# Autodesk Inventor assembly: FULL FINGE6
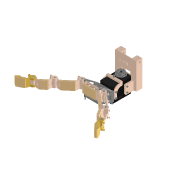
[picture p0: Inventor's stored thumbnail of the model, 180x180]
Saved by Autodesk Inventor 2021 (Build 250183000, 183)
## iProperties
Created: 2022-10-03
Part Number: FULL FINGE6
Document SubType Name: Assembly
Designer: ereg140
Author: ereg140
## Documents named in this file (21)
- \\files.auckland.ac.nz\myhome\Documents\GitHub\hand\FULL FINGE7.iam
- \\files.auckland.ac.nz\myhome\Documents\GitHub\hand\XM430 Motor\XM430-Working-Shaft.iam
- \\files.auckland.ac.nz\myhome\Documents\GitHub\hand\Dovetail\dovetail_female_Dyna_Mount.ipt
- \\files.auckland.ac.nz\myhome\Documents\GitHub\hand\Tendon_Center.ipt
- \\files.auckland.ac.nz\myhome\Documents\GitHub\hand\PLANGE7\Phalalnge7_HDM_45mm.ipt
- \\files.auckland.ac.nz\myhome\Documents\GitHub\hand\PLANGE7\Phalalnge7_HDM_35mm.ipt
- \\files.auckland.ac.nz\myhome\Documents\GitHub\hand\PLANGE7\Phalalnge7_35mm_TIP_hdm.ipt
- \\files.auckland.ac.nz\myhome\Documents\GitHub\hand\PLANGE7\FINGIE_7_palm_50mm.ipt
- \\files.auckland.ac.nz\myhome\Documents\GitHub\hand\Dynamixel_Palm_Bracket_3.ipt
- \\files.auckland.ac.nz\myhome\Documents\GitHub\hand\hardware\m2_18mm.ipt
- \\files.auckland.ac.nz\myhome\Documents\GitHub\hand\hardware\m2_40mm.ipt
- \\files.auckland.ac.nz\myhome\Documents\GitHub\hand\hardware\m2_nut.ipt
- \\files.auckland.ac.nz\myhome\Documents\GitHub\hand\hardware\M2_6mm.ipt
- \\files.auckland.ac.nz\myhome\Documents\GitHub\hand\hardware\M2_5_6mm.ipt
- \\files.auckland.ac.nz\myhome\Documents\GitHub\hand\Pully_smallest.ipt
- \\files.auckland.ac.nz\myhome\Documents\GitHub\hand\hardware\M2_3mm.ipt
- \\files.auckland.ac.nz\myhome\Documents\GitHub\hand\hardware\paperclip16mm.ipt
- \\files.auckland.ac.nz\myhome\Documents\GitHub\hand\HDM_represent\flange7-42mm.ipt
- \\files.auckland.ac.nz\myhome\Documents\GitHub\hand\HDM_represent\flange7-35mm.ipt
- \\files.auckland.ac.nz\myhome\Documents\GitHub\hand\HDM_represent\flange7-tip.ipt
- \\files.auckland.ac.nz\myhome\Documents\GitHub\hand\HDM_represent\flange7-PALM.ipt
## Components (62 placed, 20 different names)
1. XM430-Working-Shaft:1 [sub-assembly] — Mate:1, Mate:2, Slider:1, Rigid:7, Rigid:8, Rotational:1
2. dovetail_female_Dyna_Mount:1 — Mate:1, Mate:2, Slider:1, Rigid:31, Rigid:32, Rigid:35, Rigid:36
3. Dynamixel_Palm_Bracket_3:1 — Rigid:7, Rigid:9, Rigid:17, Rigid:18, Rigid:19, Rigid:20, Rigid:27, Rigid:28, Rigid:42, Rigid:43, Rigid:44, Rigid:45
4. Tendon_Center:1 — Rigid:8, Rigid:29, Rigid:30, Rigid:33, Rigid:34, Rigid:41
5. FINGIE_7_palm_50mm:1 — Rigid:9, Planar:4, Cylindrical:7, Cylindrical:12, Planar:9, Rigid:61
6. Phalalnge7_35mm_TIP_hdm:2 — Planar:6, Cylindrical:9, Rigid:11, Rigid:22, Rigid:60
7. Phalalnge7_HDM_35mm:2 — Planar:5, Planar:6, Cylindrical:8, Cylindrical:9, Rigid:10, Rigid:21, Rigid:52, Rigid:53, Rigid:58
8. Phalalnge7_HDM_45mm:2 — Planar:4, Planar:5, Cylindrical:7, Cylindrical:8, Rigid:12, Rigid:23, Rigid:50, Rigid:51, Rigid:56
9. Phalalnge7_35mm_TIP_hdm:3 — Cylindrical:11, Rigid:15, Rigid:26, Rigid:59
10. Phalalnge7_HDM_35mm:3 — Cylindrical:10, Cylindrical:11, Rigid:14, Rigid:25, Rigid:48, Rigid:49, Rigid:57
11. Phalalnge7_HDM_45mm:3 — Cylindrical:10, Cylindrical:12, Planar:9, Rigid:13, Rigid:24, Rigid:46, Rigid:47, Rigid:55
12. m2_18mm:1 — Rigid:13
13. m2_18mm:2 — Rigid:14
14. m2_18mm:3 — Rigid:10
15. m2_18mm:4 — Rigid:15
16. m2_18mm:5 — Rigid:11
17. m2_18mm:6 — Rigid:12
18. m2_40mm:1 — Rigid:19
19. m2_40mm:2 — Rigid:17
20. m2_nut:1 — Rigid:20
21. m2_nut:2 — Rigid:18
22. m2_nut:3 — Rigid:23
23. m2_nut:4 — Rigid:22
24. m2_nut:5 — Rigid:21
25. m2_nut:6 — Rigid:26
26. m2_nut:7 — Rigid:25
27. m2_nut:8 — Rigid:24
28. M2_6mm:1 — Rigid:28
29. M2_6mm:2 — Rigid:27
30. M2_5_6mm:1 — Rigid:35
31. M2_5_6mm:2 — Rigid:30
32. M2_5_6mm:3 — Rigid:34
33. M2_5_6mm:4 — Rigid:33
34. M2_5_6mm:5 — Rigid:32
35. M2_5_6mm:6 — Rigid:31
36. M2_5_6mm:8 — Rigid:29
37. M2_5_6mm:9 — Rigid:36
38. Pully_smallest:1 — Rotational:1, Rigid:37, Rigid:38, Rigid:39, Rigid:40
39. M2_3mm:1 — Rigid:39
40. M2_3mm:2 — Rigid:37
41. M2_3mm:3 — Rigid:38
42. M2_3mm:4 — Rigid:40
43. M2_6mm:3 — Rigid:41
44. M2_5_6mm:10 — Rigid:45
45. M2_5_6mm:11 — Rigid:44
46. M2_5_6mm:12 — Rigid:43
47. M2_5_6mm:13 — Rigid:42
48. paperclip16mm:1 — Rigid:51
49. paperclip16mm:2 — Rigid:52
50. paperclip16mm:3 — Rigid:53
51. paperclip16mm:4 — Rigid:49
52. paperclip16mm:5 — Rigid:48
53. paperclip16mm:6 — Rigid:50
54. paperclip16mm:7 — Rigid:46
55. paperclip16mm:8 — Rigid:47
56. flange7-42mm:1 — Rigid:56
57. flange7-42mm:2 — Rigid:55
58. flange7-35mm:1 — Rigid:57
59. flange7-35mm:2 — Rigid:58
60. flange7-tip:1 — Rigid:59
61. flange7-tip:2 — Rigid:60
62. flange7-PALM:1 — Rigid:61
## Relationships (69: WeldJoint 53, PlanarJoint 6, CylindricalJoint 6, Mate 2, TranslationJoint 1, RevoluteJoint 1)
- Mate:1: XM430-Working-Shaft:1 ↔ dovetail_female_Dyna_Mount:1
- Mate:2: XM430-Working-Shaft:1 ↔ dovetail_female_Dyna_Mount:1
- Slider:1 [TranslationJoint]: XM430-Working-Shaft:1 ↔ dovetail_female_Dyna_Mount:1
- Rigid:7 [WeldJoint]: XM430-Working-Shaft:1 ↔ Dynamixel_Palm_Bracket_3:1
- Rigid:8 [WeldJoint]: XM430-Working-Shaft:1 ↔ Tendon_Center:1
- Rigid:9 [WeldJoint]: Dynamixel_Palm_Bracket_3:1 ↔ FINGIE_7_palm_50mm:1
- Planar:4: FINGIE_7_palm_50mm:1 ↔ Phalalnge7_HDM_45mm:2
- Planar:5: Phalalnge7_HDM_35mm:2 ↔ Phalalnge7_HDM_45mm:2
- Planar:6: Phalalnge7_35mm_TIP_hdm:2 ↔ Phalalnge7_HDM_35mm:2
- Cylindrical:7: FINGIE_7_palm_50mm:1 ↔ Phalalnge7_HDM_45mm:2
- Cylindrical:8: Phalalnge7_HDM_35mm:2 ↔ Phalalnge7_HDM_45mm:2
- Cylindrical:9: Phalalnge7_35mm_TIP_hdm:2 ↔ Phalalnge7_HDM_35mm:2
- [PlanarJoint]: Phalalnge7_HDM_35mm:3 ↔ Phalalnge7_HDM_45mm:3
- [PlanarJoint]: Phalalnge7_35mm_TIP_hdm:3 ↔ Phalalnge7_HDM_35mm:3
- Cylindrical:10: Phalalnge7_HDM_35mm:3 ↔ Phalalnge7_HDM_45mm:3
- Cylindrical:11: Phalalnge7_35mm_TIP_hdm:3 ↔ Phalalnge7_HDM_35mm:3
- Cylindrical:12: FINGIE_7_palm_50mm:1 ↔ Phalalnge7_HDM_45mm:3
- Planar:9: FINGIE_7_palm_50mm:1 ↔ Phalalnge7_HDM_45mm:3
- Rigid:10 [WeldJoint]: Phalalnge7_HDM_35mm:2 ↔ m2_18mm:3
- Rigid:11 [WeldJoint]: Phalalnge7_35mm_TIP_hdm:2 ↔ m2_18mm:5
- Rigid:12 [WeldJoint]: Phalalnge7_HDM_45mm:2 ↔ m2_18mm:6
- Rigid:13 [WeldJoint]: Phalalnge7_HDM_45mm:3 ↔ m2_18mm:1
- Rigid:14 [WeldJoint]: Phalalnge7_HDM_35mm:3 ↔ m2_18mm:2
- Rigid:15 [WeldJoint]: Phalalnge7_35mm_TIP_hdm:3 ↔ m2_18mm:4
- Rigid:17 [WeldJoint]: Dynamixel_Palm_Bracket_3:1 ↔ m2_40mm:2
- Rigid:18 [WeldJoint]: Dynamixel_Palm_Bracket_3:1 ↔ m2_nut:2
- Rigid:19 [WeldJoint]: Dynamixel_Palm_Bracket_3:1 ↔ m2_40mm:1
- Rigid:20 [WeldJoint]: Dynamixel_Palm_Bracket_3:1 ↔ m2_nut:1
- Rigid:21 [WeldJoint]: Phalalnge7_HDM_35mm:2 ↔ m2_nut:5
- Rigid:22 [WeldJoint]: Phalalnge7_35mm_TIP_hdm:2 ↔ m2_nut:4
- Rigid:23 [WeldJoint]: Phalalnge7_HDM_45mm:2 ↔ m2_nut:3
- Rigid:24 [WeldJoint]: Phalalnge7_HDM_45mm:3 ↔ m2_nut:8
- Rigid:25 [WeldJoint]: Phalalnge7_HDM_35mm:3 ↔ m2_nut:7
- Rigid:26 [WeldJoint]: Phalalnge7_35mm_TIP_hdm:3 ↔ m2_nut:6
- Rigid:27 [WeldJoint]: Dynamixel_Palm_Bracket_3:1 ↔ M2_6mm:2
- Rigid:28 [WeldJoint]: Dynamixel_Palm_Bracket_3:1 ↔ M2_6mm:1
- Rigid:29 [WeldJoint]: Tendon_Center:1 ↔ M2_5_6mm:8
- Rigid:30 [WeldJoint]: Tendon_Center:1 ↔ M2_5_6mm:2
- Rigid:31 [WeldJoint]: dovetail_female_Dyna_Mount:1 ↔ M2_5_6mm:6
- Rigid:32 [WeldJoint]: dovetail_female_Dyna_Mount:1 ↔ M2_5_6mm:5
- Rigid:33 [WeldJoint]: Tendon_Center:1 ↔ M2_5_6mm:4
- Rigid:34 [WeldJoint]: Tendon_Center:1 ↔ M2_5_6mm:3
- Rigid:35 [WeldJoint]: dovetail_female_Dyna_Mount:1 ↔ M2_5_6mm:1
- Rigid:36 [WeldJoint]: dovetail_female_Dyna_Mount:1 ↔ M2_5_6mm:9
- Rotational:1 [RevoluteJoint]: XM430-Working-Shaft:1 ↔ Pully_smallest:1
- Rigid:37 [WeldJoint]: Pully_smallest:1 ↔ M2_3mm:2
- Rigid:38 [WeldJoint]: Pully_smallest:1 ↔ M2_3mm:3
- Rigid:39 [WeldJoint]: Pully_smallest:1 ↔ M2_3mm:1
- Rigid:40 [WeldJoint]: Pully_smallest:1 ↔ M2_3mm:4
- Rigid:41 [WeldJoint]: Tendon_Center:1 ↔ M2_6mm:3
- Rigid:42 [WeldJoint]: Dynamixel_Palm_Bracket_3:1 ↔ M2_5_6mm:13
- Rigid:43 [WeldJoint]: Dynamixel_Palm_Bracket_3:1 ↔ M2_5_6mm:12
- Rigid:44 [WeldJoint]: Dynamixel_Palm_Bracket_3:1 ↔ M2_5_6mm:11
- Rigid:45 [WeldJoint]: Dynamixel_Palm_Bracket_3:1 ↔ M2_5_6mm:10
- Rigid:46 [WeldJoint] (1 mm): Phalalnge7_HDM_45mm:3 ↔ paperclip16mm:7
- Rigid:47 [WeldJoint] (1 mm): Phalalnge7_HDM_45mm:3 ↔ paperclip16mm:8
- Rigid:48 [WeldJoint] (1 mm): Phalalnge7_HDM_35mm:3 ↔ paperclip16mm:5
- Rigid:49 [WeldJoint] (1 mm): Phalalnge7_HDM_35mm:3 ↔ paperclip16mm:4
- Rigid:50 [WeldJoint] (1 mm): Phalalnge7_HDM_45mm:2 ↔ paperclip16mm:6
- Rigid:51 [WeldJoint] (1 mm): Phalalnge7_HDM_45mm:2 ↔ paperclip16mm:1
- Rigid:52 [WeldJoint] (1 mm): Phalalnge7_HDM_35mm:2 ↔ paperclip16mm:2
- Rigid:53 [WeldJoint] (1 mm): Phalalnge7_HDM_35mm:2 ↔ paperclip16mm:3
- Rigid:55 [WeldJoint]: Phalalnge7_HDM_45mm:3 ↔ flange7-42mm:2
- Rigid:56 [WeldJoint]: Phalalnge7_HDM_45mm:2 ↔ flange7-42mm:1
- Rigid:57 [WeldJoint]: Phalalnge7_HDM_35mm:3 ↔ flange7-35mm:1
- Rigid:58 [WeldJoint]: Phalalnge7_HDM_35mm:2 ↔ flange7-35mm:2
- Rigid:59 [WeldJoint]: Phalalnge7_35mm_TIP_hdm:3 ↔ flange7-tip:1
- Rigid:60 [WeldJoint]: Phalalnge7_35mm_TIP_hdm:2 ↔ flange7-tip:2
- Rigid:61 [WeldJoint]: FINGIE_7_palm_50mm:1 ↔ flange7-PALM:1
## Named parameters: sa_0 = 30000, d48_d34 = 0 mm, d49_d35 = 0 mm, d50_d44 = 163.51186 deg, d51_d45 = -0.5 mm, d52_d46 = 170.025919 deg, d53_d47 = 0.5 mm
note: some values were not read from the file. Shown as the stored number, unit unknown: "sa_0".
